# Autodesk Inventor assembly: Motor mount
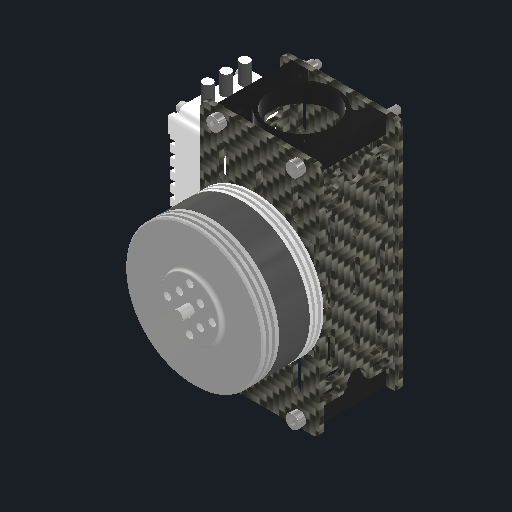
[picture p0: Inventor's stored thumbnail of the model, 512x512]
Saved by Autodesk Inventor 2025 (Build 290162010, 162A)
## iProperties
Created: 2023-12-07
Part Number: Motor mount
Document SubType Name: Assembly
Designer: dzw04
Sending System: Autodesk Translation Framework v12.14.0.127
Preprocessor: ST-DEVELOPER v20
Title: Motor mount v12.step
## Documents named in this file (10)
- C:\Users\dhrzw\OneDrive - Saxion\Sarax_Pack_And_Go\Workspaces\Workspace\SARAX\01. CAD\01. 3D_Drawing\02. Sub_Assemblies\Arm\02. Sub_Assemblies\Motor mount v12.iam
- C:\Users\dhrzw\OneDrive - Saxion\Sarax_Pack_And_Go\Workspaces\Workspace\SARAX\01. CAD\01. 3D_Drawing\02. Sub_Assemblies\Arm\01. Parts\25mm bracket v4.ipt
- C:\Users\dhrzw\OneDrive - Saxion\Sarax_Pack_And_Go\Workspaces\Workspace\SARAX\01. CAD\01. 3D_Drawing\02. Sub_Assemblies\Arm\01. Parts\ESC_Mount.ipt
- C:\Users\dhrzw\OneDrive - Saxion\Sarax_Pack_And_Go\Workspaces\Workspace\SARAX\01. CAD\01. 3D_Drawing\02. Sub_Assemblies\Arm\02. Sub_Assemblies\T motor MN501-S v2.iam
- C:\Users\dhrzw\OneDrive - Saxion\Sarax_Pack_And_Go\Workspaces\Workspace\SARAX\01. CAD\01. 3D_Drawing\02. Sub_Assemblies\Arm\02. Sub_Assemblies\T motor MN501-S v2_1.iam
- C:\Users\dhrzw\OneDrive - Saxion\Sarax_Pack_And_Go\Workspaces\Workspace\SARAX\01. CAD\01. 3D_Drawing\02. Sub_Assemblies\Arm\02. Sub_Assemblies\ESC ALPHA 60A HV Tmotor V2 v4.iam
- C:\Users\dhrzw\OneDrive - Saxion\Sarax_Pack_And_Go\Workspaces\Workspace\SARAX\01. CAD\01. 3D_Drawing\02. Sub_Assemblies\Arm\02. Sub_Assemblies\ESC ALPHA 60A HV Tmotor V2 v4_1.iam
- C:\Users\dhrzw\OneDrive - Saxion\Sarax_Pack_And_Go\Workspaces\Workspace\SARAX\01. CAD\01. 3D_Drawing\01. Parts\en-US\ISO 4762(2)\ISO 4762 - M3 x 40ISO.ipt
- C:\Users\dhrzw\OneDrive - Saxion\Sarax_Pack_And_Go\Workspaces\Workspace\SARAX\01. CAD\01. 3D_Drawing\01. Parts\en-US\ISO 10511\ISO 10511 - M3.ipt
- C:\Users\dhrzw\OneDrive - Saxion\Sarax_Pack_And_Go\Workspaces\Workspace\SARAX\01. CAD\01. 3D_Drawing\02. Sub_Assemblies\Arm\01. Parts\Motor_Mount.ipt
## Components (17 placed, 7 different names)
1. 25mm bracket v4:1 — Mate:4, Flush:3, Flush:4, Mate:6
2. 25mm bracket v4:2 — Mate:4, Flush:3, Flush:4, Mate:5, Mate:8, Mate:9
3. 25mm bracket v4:3 — Mate:3, Flush:1, Flush:2, Mate:7
4. 25mm bracket v4:4 — Mate:2, Mate:3, Flush:1, Flush:2, Mate:10, Mate:11, Mate:12
5. Component1:1 — Mate:1, Mate:2, Mate:5, Flush:5, Flush:6, Mate:8, Mate:9, Mate:10, Mate:11, Mate:15, Mate:17, Mate:18, Mate:19, Mate:20, Mate:21, Mate:22, Tangent:1
6. Component2:1 — Mate:15, Flush:7, Flush:8, Mate:19, Mate:23, Mate:24, Mate:25
7. Component1:2 — Mate:6, Mate:7, Flush:5, Flush:6, Mate:13, Angle:1, Mate:29, Mate:30, Tangent:2
8. Component2:2 — Mate:17, Flush:7, Flush:8, Mate:18, Mate:20, Mate:26, Mate:27, Mate:28
9. T motor MN501-S v2:1 [sub-assembly] — Mate:21, Mate:22, Tangent:1
10. T motor MN501-S v2:2 [sub-assembly] — Mate:29, Mate:30, Tangent:2
11. ESC ALPHA 60A HV Tmotor V2 v4:1 [sub-assembly] — Mate:26, Mate:27, Mate:28
12. ESC ALPHA 60A HV Tmotor V2 v4:2 [sub-assembly] — Mate:23, Mate:24, Mate:25
13. DIN EN ISO 10511 M3:1 — Mate:13, Mate:14, Angle:1
14. ISO 4762 M3 x 25:1 — Mate:1, Mate:12, Mate:14
15. ISO 4762 M3 x 25:2
16. ISO 4762 M3 x 25:3
17. ISO 4762 M3 x 25:4
## Component patterns: (4 elements, first: ISO 4762 M3 x 25:1)
## Relationships (40: Mate 29, Flush 8, Tangent 2, Angle 1)
- Mate:1: Component1:1 ↔ ISO 4762 M3 x 25:1
- Mate:2: 25mm bracket v4:4 ↔ Component1:1
- Mate:3: 25mm bracket v4:3 ↔ 25mm bracket v4:4
- Flush:1: 25mm bracket v4:3 ↔ 25mm bracket v4:4
- Flush:2: 25mm bracket v4:3 ↔ 25mm bracket v4:4
- Mate:4: 25mm bracket v4:1 ↔ 25mm bracket v4:2
- Flush:3: 25mm bracket v4:1 ↔ 25mm bracket v4:2
- Flush:4: 25mm bracket v4:1 ↔ 25mm bracket v4:2
- Mate:5: 25mm bracket v4:2 ↔ Component1:1
- Mate:6: 25mm bracket v4:1 ↔ Component1:2
- Mate:7: 25mm bracket v4:3 ↔ Component1:2
- Flush:5: Component1:1 ↔ Component1:2
- Flush:6: Component1:1 ↔ Component1:2
- Mate:8: 25mm bracket v4:2 ↔ Component1:1
- Mate:9: 25mm bracket v4:2 ↔ Component1:1
- Mate:10: 25mm bracket v4:4 ↔ Component1:1
- Mate:11: 25mm bracket v4:4 ↔ Component1:1
- Mate:12: 25mm bracket v4:4 ↔ ISO 4762 M3 x 25:1
- Mate:13: Component1:2 ↔ DIN EN ISO 10511 M3:1
- Mate:14: DIN EN ISO 10511 M3:1 ↔ ISO 4762 M3 x 25:1
- Angle:1 (0 deg): Component1:2 ↔ DIN EN ISO 10511 M3:1
- Mate:15: Component1:1 ↔ Component2:1
- Mate:17: Component1:1 ↔ Component2:2
- Flush:7: Component2:1 ↔ Component2:2
- Flush:8: Component2:1 ↔ Component2:2
- Mate:18: Component1:1 ↔ Component2:2
- Mate:19: Component1:1 ↔ Component2:1
- Mate:20: Component1:1 ↔ Component2:2
- Mate:21: Component1:1 ↔ T motor MN501-S v2:1
- Mate:22: Component1:1 ↔ T motor MN501-S v2:1
- Tangent:1: Component1:1 ↔ T motor MN501-S v2:1
- Mate:23: Component2:1 ↔ ESC ALPHA 60A HV Tmotor V2 v4:2
- Mate:24: Component2:1 ↔ ESC ALPHA 60A HV Tmotor V2 v4:2
- Mate:25: Component2:1 ↔ ESC ALPHA 60A HV Tmotor V2 v4:2
- Mate:26: Component2:2 ↔ ESC ALPHA 60A HV Tmotor V2 v4:1
- Mate:27: Component2:2 ↔ ESC ALPHA 60A HV Tmotor V2 v4:1
- Mate:28: Component2:2 ↔ ESC ALPHA 60A HV Tmotor V2 v4:1
- Mate:29: Component1:2 ↔ T motor MN501-S v2:2
- Mate:30: Component1:2 ↔ T motor MN501-S v2:2
- Tangent:2: Component1:2 ↔ T motor MN501-S v2:2
